# Autodesk Inventor assembly: short_link
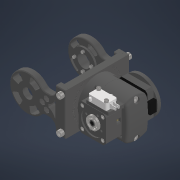
[picture p0: Inventor's stored thumbnail of the model, 180x180]
Saved by Autodesk Inventor 2022 (Build 260153070, 153G)
## iProperties
Created: 2021-11-21
Part Number: short_link
Document SubType Name: Assembly
Designer: Teo
Title: Predstavitev sklopa
Author: Teo
## Documents named in this file (16)
- D:\Zaključna\Roka\Priloge\IPT_files\Assemblies\short_link.iam
- D:\Zaključna\Roka\Priloge\IPT_files\Stepper_nema17.ipt
- D:\Zaključna\Roka\Priloge\IPT_files\Assemblies\reductor.iam
- D:\Zaključna\Roka\Priloge\IPT_files\Stepper_holder_1_lite.ipt
- D:\Zaključna\Roka\Priloge\IPT_files\Bearing_back_lite.ipt
- C:\Users\Teo\Documents\Inventor\Content Center Files\R2022\en-US\DIN 625 - T1\DIN 625 T1 - 619_8 - 8 x 19 x 6.ipt
- D:\Zaključna\Roka\Priloge\IPT_files\Forearm_short_2.ipt
- D:\Zaključna\Roka\Priloge\IPT_files\Forearm_short_1.ipt
- D:\Zaključna\Roka\Priloge\IPT_files\Stepper_bracket_1_lite.ipt
- C:\Users\Teo\Documents\Inventor\Content Center Files\R2022\en-US\DIN 912\DIN 912 - M3 x 0.5 x 25 x 18.ipt
- C:\Users\Teo\Documents\Inventor\Content Center Files\R2022\en-US\DIN 912\DIN 912 - M3 x 0.5 x 30 x 18.ipt
- C:\Users\Teo\Documents\Inventor\Content Center Files\R2022\en-US\DIN 912\DIN 912 - M4 x 0.7 x 16 x 14.25.ipt
- C:\Users\Teo\Documents\Inventor\Content Center Files\R2022\en-US\DIN 912\DIN 912 - M5 x 0.8 x 16 x 14.ipt
- C:\Users\Teo\Documents\Inventor\Content Center Files\R2022\en-US\DIN 912\DIN 912 - M5 x 0.8 x 40 x 22.ipt
- D:\Zaključna\Roka\Priloge\IPT_files\Limit_switch.ipt
- C:\Users\Teo\Documents\Inventor\Content Center Files\R2022\en-US\DIN 912\DIN 912 - M3 x 0.5 x 12 x 10.75.ipt
## Components (29 placed, 15 different names)
1. Stepper_nema17:1 — Mate:1, Mate:2, Mate:3, Mate:4, Mate:5, Mate:6, Mate:7, Mate:8, Mate:20, Mate:31, Mate:33, Mate:35, Mate:37
2. reductor:1 [sub-assembly] — Mate:1, Mate:2, Mate:3, Mate:23, Mate:24, Mate:25, Mate:26, Mate:27, Mate:28, Mate:29, Mate:30
3. Stepper_holder_1_lite:1 — Mate:4, Mate:5, Mate:11, Mate:12, Mate:13, Mate:14, Mate:15, Mate:16, Mate:17, Mate:21, Mate:22, Mate:47, Mate:49, Mate:51, Mate:53
4. Bearing_back_lite:1 — Mate:6, Mate:7, Mate:8, Mate:18, Mate:19, Mate:32, Mate:34, Mate:36, Mate:38
5. Forearm_short_2:1 — Mate:11, Mate:12, Mate:13, Mate:52, Mate:54
6. Forearm_short_1:1 — Mate:14, Mate:15, Mate:16, Mate:39, Mate:40, Mate:41, Mate:42, Mate:43, Mate:44, Mate:45, Mate:46, Mate:48, Mate:50
7. Stepper_bracket_1_lite:1 — Mate:20, Mate:21, Mate:22, Mate:55, Mate:56, Mate:57, Mate:58, Mate:59, Mate:60, Angle:1, Mate:61, Mate:63
8. Limit_switch:1 — Mate:59, Mate:60, Angle:1, Mate:62, Mate:64
9. DIN 625 - T1 619/8 - 8 x 19 x 6:1 — Mate:18, Mate:19
10. DIN 912 - replaced by DIN EN ISO 4762 M3 x 25:1 — Mate:23, Mate:24
11. DIN 912 - replaced by DIN EN ISO 4762 M3 x 25:2 — Mate:25, Mate:26
12. DIN 912 - replaced by DIN EN ISO 4762 M3 x 25:3 — Mate:27, Mate:28
13. DIN 912 - replaced by DIN EN ISO 4762 M3 x 25:4 — Mate:29, Mate:30
14. DIN 912 - replaced by DIN EN ISO 4762 M3 x 30:1 — Mate:31, Mate:32
15. DIN 912 - replaced by DIN EN ISO 4762 M3 x 30:4 — Mate:33, Mate:34
16. DIN 912 - replaced by DIN EN ISO 4762 M3 x 30:2 — Mate:35, Mate:36
17. DIN 912 - replaced by DIN EN ISO 4762 M3 x 30:3 — Mate:37, Mate:38
18. DIN 912 - replaced by DIN EN ISO 4762 M4 x 16:1 — Mate:39, Mate:40
19. DIN 912 - replaced by DIN EN ISO 4762 M4 x 16:2 — Mate:41, Mate:42
20. DIN 912 - replaced by DIN EN ISO 4762 M4 x 16:3 — Mate:43, Mate:44
21. DIN 912 - replaced by DIN EN ISO 4762 M4 x 16:4 — Mate:45, Mate:46
22. DIN 912 - replaced by DIN EN ISO 4762 M5 x 16:1 — Mate:47, Mate:48
23. DIN 912 - replaced by DIN EN ISO 4762 M5 x 16:2 — Mate:49, Mate:50
24. DIN 912 - replaced by DIN EN ISO 4762 M5 x 16:4 — Mate:51, Mate:52
25. DIN 912 - replaced by DIN EN ISO 4762 M5 x 16:3 — Mate:53, Mate:54
26. DIN 912 - replaced by DIN EN ISO 4762 M5 x 40:2 — Mate:55, Mate:56
27. DIN 912 - replaced by DIN EN ISO 4762 M5 x 40:1 — Mate:57, Mate:58
28. DIN 912 - replaced by DIN EN ISO 4762 M3 x 12:1 — Mate:61, Mate:62
29. DIN 912 - replaced by DIN EN ISO 4762 M3 x 12:2 — Mate:63, Mate:64
## Relationships (63: Mate 62, Angle 1)
- Mate:1: Stepper_nema17:1 ↔ reductor:1
- Mate:2: Stepper_nema17:1 ↔ reductor:1
- Mate:3: Stepper_nema17:1 ↔ reductor:1
- Mate:4: Stepper_nema17:1 ↔ Stepper_holder_1_lite:1
- Mate:5: Stepper_nema17:1 ↔ Stepper_holder_1_lite:1
- Mate:6: Stepper_nema17:1 ↔ Bearing_back_lite:1
- Mate:7: Stepper_nema17:1 ↔ Bearing_back_lite:1
- Mate:8: Stepper_nema17:1 ↔ Bearing_back_lite:1
- Mate:11: Stepper_holder_1_lite:1 ↔ Forearm_short_2:1
- Mate:12: Stepper_holder_1_lite:1 ↔ Forearm_short_2:1
- Mate:13: Stepper_holder_1_lite:1 ↔ Forearm_short_2:1
- Mate:14: Stepper_holder_1_lite:1 ↔ Forearm_short_1:1
- Mate:15: Stepper_holder_1_lite:1 ↔ Forearm_short_1:1
- Mate:16: Stepper_holder_1_lite:1 ↔ Forearm_short_1:1
- Mate:17: Stepper_holder_1_lite:1
- Mate:18: Bearing_back_lite:1 ↔ DIN 625 - T1 619/8 - 8 x 19 x 6:1
- Mate:19: Bearing_back_lite:1 ↔ DIN 625 - T1 619/8 - 8 x 19 x 6:1
- Mate:20: Stepper_nema17:1 ↔ Stepper_bracket_1_lite:1
- Mate:21: Stepper_holder_1_lite:1 ↔ Stepper_bracket_1_lite:1
- Mate:22: Stepper_holder_1_lite:1 ↔ Stepper_bracket_1_lite:1
- Mate:23: reductor:1 ↔ DIN 912 - replaced by DIN EN ISO 4762 M3 x 25:1
- Mate:24: reductor:1 ↔ DIN 912 - replaced by DIN EN ISO 4762 M3 x 25:1
- Mate:25: reductor:1 ↔ DIN 912 - replaced by DIN EN ISO 4762 M3 x 25:2
- Mate:26: reductor:1 ↔ DIN 912 - replaced by DIN EN ISO 4762 M3 x 25:2
- Mate:27: reductor:1 ↔ DIN 912 - replaced by DIN EN ISO 4762 M3 x 25:3
- Mate:28: reductor:1 ↔ DIN 912 - replaced by DIN EN ISO 4762 M3 x 25:3
- Mate:29: reductor:1 ↔ DIN 912 - replaced by DIN EN ISO 4762 M3 x 25:4
- Mate:30: reductor:1 ↔ DIN 912 - replaced by DIN EN ISO 4762 M3 x 25:4
- Mate:31: Stepper_nema17:1 ↔ DIN 912 - replaced by DIN EN ISO 4762 M3 x 30:1
- Mate:32: Bearing_back_lite:1 ↔ DIN 912 - replaced by DIN EN ISO 4762 M3 x 30:1
- Mate:33: Stepper_nema17:1 ↔ DIN 912 - replaced by DIN EN ISO 4762 M3 x 30:4
- Mate:34: Bearing_back_lite:1 ↔ DIN 912 - replaced by DIN EN ISO 4762 M3 x 30:4
- Mate:35: Stepper_nema17:1 ↔ DIN 912 - replaced by DIN EN ISO 4762 M3 x 30:2
- Mate:36: Bearing_back_lite:1 ↔ DIN 912 - replaced by DIN EN ISO 4762 M3 x 30:2
- Mate:37: Stepper_nema17:1 ↔ DIN 912 - replaced by DIN EN ISO 4762 M3 x 30:3
- Mate:38: Bearing_back_lite:1 ↔ DIN 912 - replaced by DIN EN ISO 4762 M3 x 30:3
- Mate:39: Forearm_short_1:1 ↔ DIN 912 - replaced by DIN EN ISO 4762 M4 x 16:1
- Mate:40: Forearm_short_1:1 ↔ DIN 912 - replaced by DIN EN ISO 4762 M4 x 16:1
- Mate:41: Forearm_short_1:1 ↔ DIN 912 - replaced by DIN EN ISO 4762 M4 x 16:2
- Mate:42: Forearm_short_1:1 ↔ DIN 912 - replaced by DIN EN ISO 4762 M4 x 16:2
- Mate:43: Forearm_short_1:1 ↔ DIN 912 - replaced by DIN EN ISO 4762 M4 x 16:3
- Mate:44: Forearm_short_1:1 ↔ DIN 912 - replaced by DIN EN ISO 4762 M4 x 16:3
- Mate:45: Forearm_short_1:1 ↔ DIN 912 - replaced by DIN EN ISO 4762 M4 x 16:4
- Mate:46: Forearm_short_1:1 ↔ DIN 912 - replaced by DIN EN ISO 4762 M4 x 16:4
- Mate:47: Stepper_holder_1_lite:1 ↔ DIN 912 - replaced by DIN EN ISO 4762 M5 x 16:1
- Mate:48: Forearm_short_1:1 ↔ DIN 912 - replaced by DIN EN ISO 4762 M5 x 16:1
- Mate:49: Stepper_holder_1_lite:1 ↔ DIN 912 - replaced by DIN EN ISO 4762 M5 x 16:2
- Mate:50: Forearm_short_1:1 ↔ DIN 912 - replaced by DIN EN ISO 4762 M5 x 16:2
- Mate:51: Stepper_holder_1_lite:1 ↔ DIN 912 - replaced by DIN EN ISO 4762 M5 x 16:4
- Mate:52: Forearm_short_2:1 ↔ DIN 912 - replaced by DIN EN ISO 4762 M5 x 16:4
- Mate:53: Stepper_holder_1_lite:1 ↔ DIN 912 - replaced by DIN EN ISO 4762 M5 x 16:3
- Mate:54: Forearm_short_2:1 ↔ DIN 912 - replaced by DIN EN ISO 4762 M5 x 16:3
- Mate:55: Stepper_bracket_1_lite:1 ↔ DIN 912 - replaced by DIN EN ISO 4762 M5 x 40:2
- Mate:56: Stepper_bracket_1_lite:1 ↔ DIN 912 - replaced by DIN EN ISO 4762 M5 x 40:2
- Mate:57: Stepper_bracket_1_lite:1 ↔ DIN 912 - replaced by DIN EN ISO 4762 M5 x 40:1
- Mate:58: Stepper_bracket_1_lite:1 ↔ DIN 912 - replaced by DIN EN ISO 4762 M5 x 40:1
- Mate:59: Stepper_bracket_1_lite:1 ↔ Limit_switch:1
- Mate:60: Stepper_bracket_1_lite:1 ↔ Limit_switch:1
- Angle:1 (0 deg): Stepper_bracket_1_lite:1 ↔ Limit_switch:1
- Mate:61: Stepper_bracket_1_lite:1 ↔ DIN 912 - replaced by DIN EN ISO 4762 M3 x 12:1
- Mate:62: Limit_switch:1 ↔ DIN 912 - replaced by DIN EN ISO 4762 M3 x 12:1
- Mate:63: Stepper_bracket_1_lite:1 ↔ DIN 912 - replaced by DIN EN ISO 4762 M3 x 12:2
- Mate:64: Limit_switch:1 ↔ DIN 912 - replaced by DIN EN ISO 4762 M3 x 12:2
